# Autodesk Inventor assembly: one_wheel
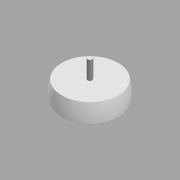
[picture p0: Inventor's stored thumbnail of the model, 180x180]
Saved by Autodesk Inventor 2021.3 (Build 253353000, 353)
## iProperties
Created: 2021-05-27
Part Number: one_wheel
Document SubType Name: Assembly
Designer: gisen
Author: gisen
## Documents named in this file (2)
- C:\Users\gisen\workspace\beetle_inventor_model\suspension\one_wheel.iam
- C:\Users\gisen\workspace\beetle_inventor_model\suspension\6inch_wheel.ipt
## Components (1 placed, 1 different names)
1. 6inch_wheel:1 — メイト:1, メイト:2
## Relationships (2: Mate 2)
- メイト:1 [Mate]: 6inch_wheel:1
- メイト:2 [Mate]: 6inch_wheel:1
